# Autodesk Inventor assembly: Final Robot assembly
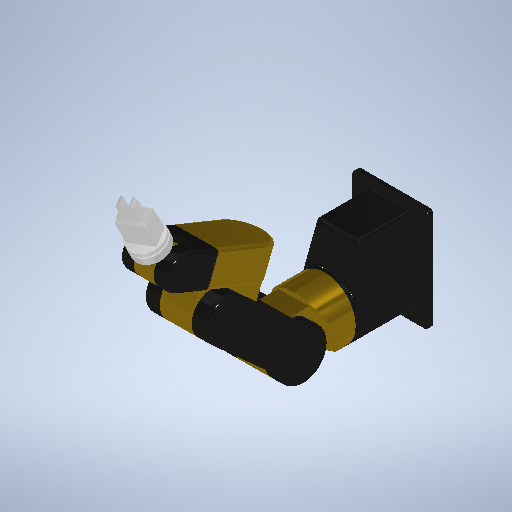
[picture p0: Inventor's stored thumbnail of the model, 512x512]
Saved by Autodesk Inventor 2025 (Build 290162000, 162)
## iProperties
Created: 2024-09-01
Part Number: Final Robot assembly
Document SubType Name: Assembly
Designer: SANDHYA
Author: SANDHYA
## Documents named in this file (9)
- C:\Users\SANDHYA\Desktop\Robotic arm\Robot Arm Assembly\Final Robot assembly.iam
- C:\Users\SANDHYA\Desktop\Robotic arm\Robot Arm Assembly\Robot-Base-Model-A.ipt
- C:\Users\SANDHYA\Desktop\Robotic arm\Robot Arm Assembly\Robot-Axis1-2.ipt
- C:\Users\SANDHYA\Desktop\Robotic arm\Robot Arm Assembly\Robot-Axis2-3.ipt
- C:\Users\SANDHYA\Desktop\Robotic arm\Robot Arm Assembly\Robot-Axis3-4.ipt
- C:\Users\SANDHYA\Desktop\Robotic arm\Robot Arm Assembly\Robot-Axis4-5.ipt
- C:\Users\SANDHYA\Desktop\Robotic arm\Robot Arm Assembly\Robot-Axis5.ipt
- C:\Users\SANDHYA\Desktop\Robotic arm\Robot Arm Assembly\Robot-Axis5-Adapter.ipt
- C:\Users\SANDHYA\Desktop\Robotic arm\Robot Arm Assembly\Robot-Gripper Assay.iam
## Components (8 placed, 8 different names)
1. Robot-Base-Model-A:1 — Mate:1, Mate:2
2. Robot-Axis1-2:1 — Mate:1, Mate:2, Mate:3, Mate:4
3. Robot-Axis2-3:1 — Mate:3, Mate:4, Mate:5, Mate:6, Angle:1
4. Robot-Axis3-4:1 — Mate:5, Mate:6, Angle:1, Mate:7, Angle:2, Angle:3
5. Robot-Axis4-5:1 — Mate:7, Angle:2, Mate:8, Flush:1, Angle:3
6. Robot-Axis5:1 — Insert:1, Mate:8, Flush:1
7. Robot-Axis5-Adapter:1 — Insert:1, Insert:2, Mate:9
8. Robot-Gripper Assay:1 [sub-assembly] — Insert:2, Mate:9
## Relationships (15: Mate 9, Angle 3, Insert 2, Flush 1)
- Mate:1: Robot-Base-Model-A:1 ↔ Robot-Axis1-2:1
- Mate:2: Robot-Base-Model-A:1 ↔ Robot-Axis1-2:1
- Mate:3: Robot-Axis1-2:1 ↔ Robot-Axis2-3:1
- Mate:4: Robot-Axis1-2:1 ↔ Robot-Axis2-3:1
- Mate:5: Robot-Axis2-3:1 ↔ Robot-Axis3-4:1
- Mate:6: Robot-Axis2-3:1 ↔ Robot-Axis3-4:1
- Angle:1 (-20 deg): Robot-Axis2-3:1 ↔ Robot-Axis3-4:1
- Mate:7: Robot-Axis3-4:1 ↔ Robot-Axis4-5:1
- Angle:2 (0 deg): Robot-Axis3-4:1 ↔ Robot-Axis4-5:1
- Insert:1: Robot-Axis5:1 ↔ Robot-Axis5-Adapter:1
- Mate:8: Robot-Axis4-5:1 ↔ Robot-Axis5:1
- Flush:1: Robot-Axis4-5:1 ↔ Robot-Axis5:1
- Insert:2: Robot-Axis5-Adapter:1 ↔ Robot-Gripper Assay:1
- Mate:9: Robot-Axis5-Adapter:1 ↔ Robot-Gripper Assay:1
- Angle:3 (0 deg): Robot-Axis3-4:1 ↔ Robot-Axis4-5:1
